# Autodesk Inventor assembly: ASSY4
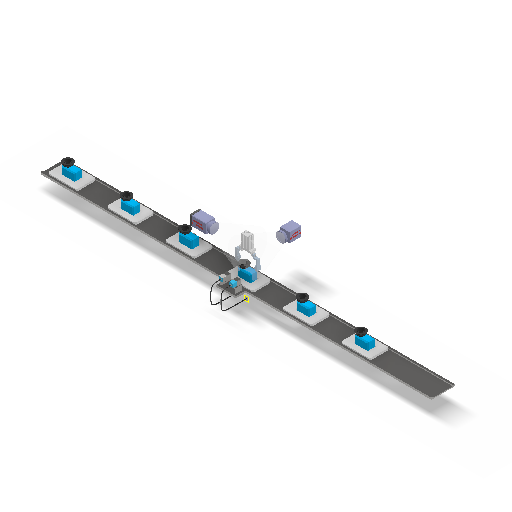
[picture p0: Inventor's stored thumbnail of the model, 512x512]
Saved by Autodesk Inventor 2025 (Build 290162000, 162)
## iProperties
Created: 2024-09-26
Part Number: ASSY4
Document SubType Name: Assembly
Designer: DMIADX
Author: DMIADX
## Documents named in this file (15)
- C:\Users\DMIADX\Documents\Inventor\chuck\ASSY4.iam
- C:\Users\DMIADX\Documents\Inventor\chuck\chuck.ipt
- C:\Users\DMIADX\Documents\Inventor\chuck\chuck_MIR.ipt
- C:\Users\DMIADX\Documents\Inventor\chuck\MHZL2-20D\MHZL2-20D.ipt
- C:\Users\DMIADX\Documents\Inventor\chuck\Connector2.ipt
- C:\Users\DMIADX\Documents\Inventor\Content Center Files\R2025\en-US\ISO 4762(2)\ISO 4762 - M3 x 12ISO.ipt
- C:\Users\DMIADX\Documents\Inventor\chuck\pallet.ipt
- C:\Users\DMIADX\Documents\Inventor\chuck\part.ipt
- C:\Users\DMIADX\Documents\Inventor\chuck\CAMERA TERMINAL.ipt
- C:\Users\DMIADX\Documents\Inventor\chuck\CAMERA.ipt
- C:\Users\DMIADX\Documents\Inventor\chuck\flash.ipt
- C:\Users\DMIADX\Documents\Inventor\chuck\jalur.ipt
- C:\Users\DMIADX\Documents\Inventor\chuck\holder sensor.ipt
- C:\Users\DMIADX\Documents\Inventor\chuck\cover.ipt
- C:\Users\DMIADX\Documents\Inventor\chuck\sensor.ipt
## Components (30 placed, 14 different names)
1. chuck:1 — Mate:3, Mate:5, Mate:6, Insert:1, Insert:2
2. chuck_MIR:1 — Mate:7, Mate:8, Mate:9, Insert:3, Insert:4, chuck naik
3. MHZL2-20D:1 — Mate:1, Mate:2, chuck 1 open, chuck 2 open, Flush:4, Flush:6
4. Connector2:1 — Flush:1, Mate:1, Mate:2, Flush:2, Mate:3, chuck 1 open, Mate:5, Mate:6
5. Connector2:2 — Flush:1, Flush:2, chuck 2 open, Mate:7, Mate:8, Mate:9
6. ISO 4762 M3 x 12:1 — Insert:1
7. ISO 4762 M3 x 12:2 — Insert:2
8. ISO 4762 M3 x 12:3 — Insert:4
9. ISO 4762 M3 x 12:4 — Insert:3
10. pallet:2 — Mate:12, Flush:12, Flush:14, Mate:24, Mate:40, Mate:41, Mate:47
11. part:2 — Mate:13, Mate:40, Mate:41, Flush:26
12. CAMERA TERMINAL:1 — Flush:16, Mate:16, Flush:17, Insert:6
13. CAMERA:1 — Flush:15, Mate:14, Mate:15, Insert:5
14. flash:1 — Insert:5
15. flash:2 — Insert:6
16. jalur:1 — Mate:17, Mate:18, Flush:18, Mate:19, Mate:23, Mate:42, Flush:19, Flush:20, Mate:45, Mate:46, Mate:53, Mate:54, Mate:59, Mate:60, Mate:65, Mate:66
17. pallet:3 — Mate:19, Mate:22, Mate:23, Mate:24, Mate:38, Mate:39, Mate:55
18. part:3 — Mate:22, Mate:38, Mate:39
19. holder sensor:1 — Mate:42, Flush:19, Flush:20, Flush:21, Mate:43, Flush:22, Flush:23, Mate:44, Flush:24, Flush:25
20. cover:1 — Mate:35, Mate:36, Mate:37
21. sensor:1 — Flush:23, Mate:44, Flush:24
22. sensor:2 — Mate:35, Mate:36, Mate:37, Flush:21, Mate:43, Flush:22, Flush:25
23. pallet:4 — Mate:45, Mate:46, Mate:47, Mate:48, Mate:49, Mate:61
24. part:4 — Mate:48, Flush:26, Mate:49
25. pallet:5 — Mate:53, Mate:54, Mate:55
26. part:5
27. pallet:6 — Mate:59, Mate:60, Mate:61, Mate:67
28. part:6
29. pallet:7 — Mate:65, Mate:66, Mate:67
30. part:7
## Relationships (79: Mate 53, Flush 20, Insert 6)
- Flush:1: Connector2:1 ↔ Connector2:2
- Mate:1: MHZL2-20D:1 ↔ Connector2:1
- Mate:2: MHZL2-20D:1 ↔ Connector2:1
- Flush:2: Connector2:1 ↔ Connector2:2
- Mate:3: chuck:1 ↔ Connector2:1
- chuck 1 open [Flush] (15.65 mm): MHZL2-20D:1 ↔ Connector2:1
- chuck 2 open [Mate] (15.65 mm): MHZL2-20D:1 ↔ Connector2:2
- Mate:5: chuck:1 ↔ Connector2:1
- Mate:6: chuck:1 ↔ Connector2:1
- Mate:7: chuck_MIR:1 ↔ Connector2:2
- Mate:8: chuck_MIR:1 ↔ Connector2:2
- Mate:9: chuck_MIR:1 ↔ Connector2:2
- Insert:1: chuck:1 ↔ ISO 4762 M3 x 12:1
- Insert:2: chuck:1 ↔ ISO 4762 M3 x 12:2
- Insert:3: chuck_MIR:1 ↔ ISO 4762 M3 x 12:4
- Insert:4: chuck_MIR:1 ↔ ISO 4762 M3 x 12:3
- Flush:4: MHZL2-20D:1
- chuck naik [Flush] (67 mm): chuck_MIR:1
- Flush:6: MHZL2-20D:1
- Mate:12: pallet:2
- Mate:13 (-8 mm): part:2
- Flush:12: pallet:2
- Flush:14 (300 mm): pallet:2
- Flush:15: CAMERA:1
- Mate:14 (-100 mm): CAMERA:1
- Mate:15 (250 mm): CAMERA:1
- Flush:16 (-30 mm): CAMERA TERMINAL:1
- Mate:16 (-110 mm): CAMERA TERMINAL:1
- Flush:17 (300 mm): CAMERA TERMINAL:1
- Insert:5: CAMERA:1 ↔ flash:1
- Insert:6: CAMERA TERMINAL:1 ↔ flash:2
- Mate:17: jalur:1
- Mate:18: jalur:1
- Flush:18: jalur:1
- Mate:19: jalur:1 ↔ pallet:3
- Mate:22: pallet:3 ↔ part:3
- Mate:23: jalur:1 ↔ pallet:3
- Mate:24 (150 mm): pallet:2 ↔ pallet:3
- Mate:35: cover:1 ↔ sensor:2
- Mate:36: cover:1 ↔ sensor:2
- Mate:37: cover:1 ↔ sensor:2
- Mate:38: pallet:3 ↔ part:3
- Mate:39: pallet:3 ↔ part:3
- Mate:40: pallet:2 ↔ part:2
- Mate:41: pallet:2 ↔ part:2
- Mate:42: jalur:1 ↔ holder sensor:1
- Flush:19: jalur:1 ↔ holder sensor:1
- Flush:20 (950 mm): jalur:1 ↔ holder sensor:1
- Flush:21: holder sensor:1 ↔ sensor:2
- Mate:43: holder sensor:1 ↔ sensor:2
- Flush:22: holder sensor:1 ↔ sensor:2
- Flush:23: holder sensor:1 ↔ sensor:1
- Mate:44: holder sensor:1 ↔ sensor:1
- Flush:24: holder sensor:1 ↔ sensor:1
- Flush:25: holder sensor:1 ↔ sensor:2
- Mate:45: jalur:1 ↔ pallet:4
- Mate:46: jalur:1 ↔ pallet:4
- Mate:47 (150 mm): pallet:2 ↔ pallet:4
- Mate:48: pallet:4 ↔ part:4
- Flush:26: part:2 ↔ part:4
- Mate:49: pallet:4 ↔ part:4
- [Mate]: pallet:5 ↔ part:5
- [Mate]: pallet:5 ↔ part:5
- [Mate]: pallet:5 ↔ part:5
- Mate:53: jalur:1 ↔ pallet:5
- Mate:54: jalur:1 ↔ pallet:5
- Mate:55 (150 mm): pallet:3 ↔ pallet:5
- [Mate]: pallet:6 ↔ part:6
- [Mate]: pallet:6 ↔ part:6
- [Mate]: pallet:6 ↔ part:6
- Mate:59: jalur:1 ↔ pallet:6
- Mate:60: jalur:1 ↔ pallet:6
- Mate:61 (150 mm): pallet:4 ↔ pallet:6
- [Mate]: pallet:7 ↔ part:7
- [Mate]: pallet:7 ↔ part:7
- [Mate]: pallet:7 ↔ part:7
- Mate:65: jalur:1 ↔ pallet:7
- Mate:66: jalur:1 ↔ pallet:7
- Mate:67 (150 mm): pallet:6 ↔ pallet:7
## Named parameters: d103_d83 = 0 mm, d104_d84 = 0 mm, d105_d58 = 0 mm, d109_d83 = 0 mm, d110_d84 = 0 mm, d111_d58 = 0 mm, d115_d83 = 0 mm, d116_d84 = 0 mm, d117_d58 = 0 mm
